# Autodesk Inventor assembly: right_leg
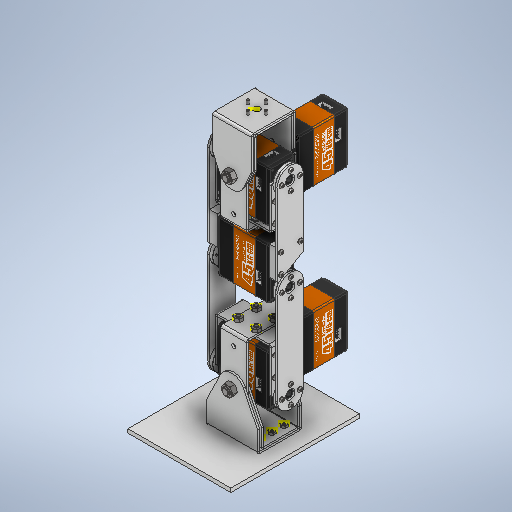
[picture p0: Inventor's stored thumbnail of the model, 512x512]
Saved by Autodesk Inventor 2026.1 (Build 301233000, 233)
## iProperties
Created: 2025-08-03
Part Number: right_leg
Document SubType Name: Assembly
Designer: User
Author: User
## Documents named in this file (29)
- C:\Users\chris\Documents\Inventor\RHp_Humanoid_ver1\Total\right_leg.iam
- C:\Users\chris\Documents\Inventor\RHp_Humanoid_ver1\Part_Body\HTD-45H, Horn (Silver)\HTD-45H\HTD-45H.iam
- C:\Users\chris\Documents\Inventor\RHp_Humanoid_ver1\Part_Leg\Frame\Leg\Left Leg\axis_1_top_frame.ipt
- C:\Users\chris\Documents\Inventor\RHp_Humanoid_ver1\Part_Leg\Frame\Leg\Left Leg\axis_3_bottom_frame.ipt
- C:\Users\chris\Documents\Inventor\RHp_Humanoid_ver1\Part_Leg\Frame\Leg\Left Leg\axis_2_bottom_frame.ipt
- C:\Users\chris\Documents\Inventor\RHp_Humanoid_ver1\Part_Leg\Frame\Leg\Left Leg\axis_1_supplement_frame.ipt
- C:\Users\chris\Documents\Inventor\RHp_Humanoid_ver1\Part_Leg\Frame\Leg\Left Leg\axis_2_4_connector_frame_powered.ipt
- C:\Users\chris\Documents\Inventor\RHp_Humanoid_ver1\Part_Leg\Frame\Leg\Left Leg\axis_2_4_connector_frame_non_powered.ipt
- C:\Users\chris\Documents\Inventor\RHp_Humanoid_ver1\Part_Leg\Frame\Leg\3D_printed_part_powered.ipt
- C:\Users\chris\Documents\Inventor\RHp_Humanoid_ver1\Part_Leg\Frame\Leg\3D_printed_part_non_powered.ipt
- C:\Users\chris\Documents\Inventor\RHp_Humanoid_ver1\Part_Leg\Frame\Leg\Left Leg\axis_4_5_connector_frame_powered.ipt
- C:\Users\chris\Documents\Inventor\RHp_Humanoid_ver1\Part_Leg\Frame\Leg\Left Leg\axis_4_5_connector_frame_non_powered.ipt
- C:\Users\chris\Documents\Inventor\RHp_Humanoid_ver1\Part_Leg\Frame\Leg\Left Leg\axis_5_top_frame.ipt
- C:\Users\chris\Documents\Inventor\RHp_Humanoid_ver1\Part_Leg\Frame\Leg\Left Leg\axis_6_top_frame.ipt
- C:\Users\chris\Documents\Inventor\RHp_Humanoid_ver1\Part_Leg\Frame\Leg\Left Leg\axis_6_bottom_frame(top).ipt
- C:\Users\chris\Documents\Inventor\RHp_Humanoid_ver1\Part_Leg\Frame\Leg\Left Leg\axis_6_bottom_frame(bottom).ipt
- C:\Users\chris\Documents\Inventor\RHp_Humanoid_ver1\Part_Leg\Frame\Leg\Left Leg\axis_6_supplement_frame.ipt
- C:\Users\chris\Documents\Inventor\RHp_Humanoid_ver1\Part_Leg\Bolt, Bearing, Nut, Washer\볼트, 너트\볼트, 너트\M5x10 Bolt.ipt
- C:\Users\chris\Documents\Inventor\RHp_Humanoid_ver1\Part_Leg\Bolt, Bearing, Nut, Washer\볼트, 너트\볼트, 너트\M5 Nylon Nut.ipt
- C:\Users\chris\Documents\Inventor\RHp_Humanoid_ver1\Part_Leg\Bolt, Bearing, Nut, Washer\볼트, 너트\볼트, 너트\M3x6 Bolt.ipt
- C:\Users\chris\Documents\Inventor\RHp_Humanoid_ver1\Part_Leg\Bolt, Bearing, Nut, Washer\볼트, 너트\볼트, 너트\M3 Nut.ipt
- C:\Users\chris\Documents\Inventor\RHp_Humanoid_ver1\Part_Leg\Bolt, Bearing, Nut, Washer\볼트, 너트\볼트, 너트\M2x6 Bolt.ipt
- C:\Users\chris\Documents\Inventor\RHp_Humanoid_ver1\Part_Leg\Bolt, Bearing, Nut, Washer\볼트, 너트\볼트, 너트\M2x4 Bolt.ipt
- C:\Users\chris\Documents\Inventor\RHp_Humanoid_ver1\Part_Leg\Bolt, Bearing, Nut, Washer\볼트, 너트\볼트, 너트\M2x12 Bolt.ipt
- C:\Users\chris\Documents\Inventor\RHp_Humanoid_ver1\Part_Leg\Bolt, Bearing, Nut, Washer\볼트, 너트\볼트, 너트\M2x8접시.ipt
- C:\Users\chris\Documents\Inventor\RHp_Humanoid_ver1\Part_Leg\Bolt, Bearing, Nut, Washer\볼트, 너트\볼트, 너트\M2x45 Bolt.ipt
- C:\Users\chris\Documents\Inventor\RHp_Humanoid_ver1\Part_Leg\HTD-45H, Horn (Silver)\HTD-45H, Horn (Silver)\Horn\Top Horn.ipt
- C:\Users\chris\Documents\Inventor\RHp_Humanoid_ver1\Part_Leg\HTD-45H, Horn (Silver)\HTD-45H, Horn (Silver)\Horn\Bottom Horn.ipt
- C:\Users\chris\Documents\Inventor\RHp_Humanoid_ver1\Part_Leg\Bolt, Bearing, Nut, Washer\M2 Nut.ipt
## Components (132 placed, 28 different names)
1. axis_1_top_frame:1 — Rigid:2, Rigid:7, Rigid:14
2. axis_1_supplement_frame:1 — Rigid:2, Rigid:3, Rigid:4, Rigid:5, Rigid:6, Rigid:8, Rigid:9, Rigid:10, Rigid:11, Rigid:13
3. HTD-45H:3 [sub-assembly] — Rigid:15, Rotational:3
4. Top Horn:2 — Rotational:3, Rigid:17
5. Bottom Horn:2 — Rigid:27
6. axis_2_bottom_frame:1 — Rigid:15, Rigid:16, Rigid:22, Rigid:23, Rigid:24, Rigid:25, Rigid:26, Rigid:28, Rigid:29, Rigid:30, Rigid:31, Rigid:40, Rigid:41, Rigid:42, Rigid:43
7. axis_2_4_connector_frame_powered:1 — Rigid:17, Rigid:18, Rigid:19, Rigid:20, Rigid:21, Rigid:55, Rigid:56, Rigid:57, Rigid:58, Rigid:59, Rigid:60
8. axis_2_4_connector_frame_non_powered:1 — Rigid:27, Rigid:32, Rigid:33, Rigid:50, Rigid:34, Rigid:49, Rigid:51, Rigid:52, Rigid:53
9. HTD-45H:2 [sub-assembly] — Rotational:2, Rigid:12
10. Top Horn:3 — Rotational:2, Rigid:7
11. axis_3_bottom_frame:1 — Rigid:12, Rigid:16, Rigid:35, Rigid:36, Rigid:37, Rigid:38, Rigid:39, Rigid:44, Rigid:45, Rigid:46, Rigid:47
12. HTD-45H:4 [sub-assembly] — Rigid:48, Rigid:54, Rotational:4, Rotational:5
13. Top Horn:4 — Rotational:4, Rigid:61
14. Bottom Horn:4 — Rotational:5, Rigid:66
15. 3D_printed_part_powered:1 — Rigid:54, Rigid:55
16. 3D_printed_part_non_powered:1 — Rigid:48, Rigid:49
17. axis_4_5_connector_frame_powered:1 — Rigid:61, Rigid:62, Rigid:63, Rigid:64, Rigid:65, Rigid:81, Rigid:82, Rigid:83, Rigid:84, Rigid:106
18. axis_4_5_connector_frame_non_powered:1 — Rigid:66, Rigid:67, Rigid:68, Rigid:69, Rigid:70, Rigid:109, Rigid:90, Rigid:91, Rigid:92, Rigid:93
19. HTD-45H:5 [sub-assembly] — Rotational:6, Rotational:7, Rigid:127
20. Top Horn:5 — Rotational:6, Rigid:106
21. Bottom Horn:5 — Rotational:7, Rigid:109
22. axis_5_top_frame:1 — Rigid:72, Rigid:73, Rigid:74, Rigid:75, Rigid:76, Rigid:85, Rigid:86, Rigid:87, Rigid:88, Rigid:89, Rigid:110, Rigid:111, Rigid:112, Rigid:113, Rigid:127
23. HTD-45H:6 [sub-assembly] — Rigid:94, Rotational:8
24. Top Horn:6 — Rotational:8, Rigid:100
25. axis_6_top_frame:1 — Rigid:72, Rigid:77, Rigid:78, Rigid:79, Rigid:80, Rigid:94, Rigid:95, Rigid:96, Rigid:97, Rigid:98, Rigid:99
26. axis_6_supplement_frame:1 — Rigid:101, Rigid:102, Rigid:103, Rigid:104, Rigid:105, Rigid:107, Rigid:121, Rigid:122, Rigid:123, Rigid:124, Rigid:125, Rigid:126
27. axis_6_bottom_frame(top):1 — Rigid:100, Rigid:101, Rigid:108, Rigid:114
28. axis_6_bottom_frame(bottom):1 — Rigid:114, Rigid:115, Rigid:116, Rigid:117, Rigid:118, Rigid:119, Rigid:120
29. M2x4 Bolt:1 — Rigid:81
30. M2x4 Bolt:2 — Rigid:82
31. M2x4 Bolt:3 — Rigid:83
32. M2x4 Bolt:4 — Rigid:84
33. M2x4 Bolt:5 — Rigid:62
34. M2x4 Bolt:6 — Rigid:63
35. M2x4 Bolt:7 — Rigid:64
36. M2x4 Bolt:8 — Rigid:65
37. M2x4 Bolt:9 — Rigid:18
38. M2x4 Bolt:10 — Rigid:19
39. M2x4 Bolt:11 — Rigid:20
40. M2x4 Bolt:12 — Rigid:21
41. M2x4 Bolt:13 — Rigid:90
42. M2x4 Bolt:14 — Rigid:91
43. M2x4 Bolt:15 — Rigid:92
44. M2x4 Bolt:16 — Rigid:93
45. M2x4 Bolt:17 — Rigid:67
46. M2x4 Bolt:18 — Rigid:68
47. M2x4 Bolt:19 — Rigid:69
48. M2x4 Bolt:20 — Rigid:70
49. M2x4 Bolt:21 — Rigid:32
50. M2x4 Bolt:22 — Rigid:33
51. M2x4 Bolt:23 — Rigid:50
52. M2x4 Bolt:24 — Rigid:34
53. M2x6 Bolt:1 — Rigid:85
54. M2x6 Bolt:2 — Rigid:86
55. M2x6 Bolt:3 — Rigid:87
56. M2x6 Bolt:4 — Rigid:88
57. M2x6 Bolt:5 — Rigid:89
58. M2x6 Bolt:6 — Rigid:110
59. M2x6 Bolt:7 — Rigid:111
60. M2x6 Bolt:8 — Rigid:112
61. M2x6 Bolt:9 — Rigid:113
62. M2x6 Bolt:10 — Rigid:95
63. M2x6 Bolt:11 — Rigid:96
64. M2x6 Bolt:12 — Rigid:99
65. M2x6 Bolt:13 — Rigid:97
66. M2x6 Bolt:14 — Rigid:98
67. M2x6 Bolt:15 — Rigid:26
68. M2x6 Bolt:16 — Rigid:25
69. M2x6 Bolt:17 — Rigid:24
70. M2x6 Bolt:18 — Rigid:23
71. M2x6 Bolt:19 — Rigid:22
72. M2x6 Bolt:20 — Rigid:28
73. M2x6 Bolt:21 — Rigid:29
74. M2x6 Bolt:22 — Rigid:30
75. M2x6 Bolt:23 — Rigid:31
76. M2x6 Bolt:24 — Rigid:39
77. M2x6 Bolt:25 — Rigid:38
78. M2x6 Bolt:26 — Rigid:37
79. M2x6 Bolt:27 — Rigid:36
80. M2x6 Bolt:28 — Rigid:35
81. M2x6 Bolt:29 — Rigid:102
82. M2x6 Bolt:30 — Rigid:103
83. M2x6 Bolt:31 — Rigid:104
84. M2x6 Bolt:32 — Rigid:105
85. M2x6 Bolt:33 — Rigid:8
86. M2x6 Bolt:34 — Rigid:9
87. M2x6 Bolt:35 — Rigid:10
88. M2x6 Bolt:36 — Rigid:11
89. M2x6 Bolt:37 — Rigid:4
90. M2x6 Bolt:38 — Rigid:5
91. M2x6 Bolt:39 — Rigid:6
92. M2x6 Bolt:40 — Rigid:3
93. M2x8접시:1 — Rigid:115
94. M2x8접시:2 — Rigid:116
95. M2x8접시:3 — Rigid:117
96. M2x8접시:4 — Rigid:118
97. M2x8접시:5 — Rigid:119
98. M2x8접시:6 — Rigid:120
99. M2x12 Bolt:1 — Rigid:58
100. M2x12 Bolt:2 — Rigid:59
101. M2x12 Bolt:3 — Rigid:60
102. M2x12 Bolt:4 — Rigid:51
103. M2x12 Bolt:5 — Rigid:52
104. M2x12 Bolt:6 — Rigid:53
105. M2x45 Bolt:1 — Rigid:56
106. M2x45 Bolt:2 — Rigid:57
107. M2 Nut:1 — Rigid:121
108. M2 Nut:2 — Rigid:122
109. M2 Nut:3 — Rigid:123
110. M2 Nut:4 — Rigid:124
111. M2 Nut:5 — Rigid:125
112. M2 Nut:6 — Rigid:126
113. M3x6 Bolt:1 — Rigid:40
114. M3x6 Bolt:2 — Rigid:42
115. M3x6 Bolt:3 — Rigid:41
116. M3x6 Bolt:4 — Rigid:43
117. M3x6 Bolt:5 — Rigid:73
118. M3x6 Bolt:6 — Rigid:75
119. M3x6 Bolt:7 — Rigid:74
120. M3x6 Bolt:8 — Rigid:76
121. M3 Nut:1 — Rigid:46
122. M3 Nut:2 — Rigid:44
123. M3 Nut:3 — Rigid:45
124. M3 Nut:4 — Rigid:47
125. M3 Nut:5 — Rigid:77
126. M3 Nut:6 — Rigid:78
127. M3 Nut:7 — Rigid:79
128. M3 Nut:8 — Rigid:80
129. M5x10 Bolt:1 — Rigid:13
130. M5x10 Bolt:4 — Rigid:107
131. M5 Nylon Nut:1 — Rigid:14
132. M5 Nylon Nut:2 — Rigid:108
## Relationships (132: WeldJoint 125, RevoluteJoint 7)
- Rigid:2 [WeldJoint]: axis_1_top_frame:1 ↔ axis_1_supplement_frame:1
- Rigid:3 [WeldJoint]: axis_1_supplement_frame:1 ↔ M2x6 Bolt:40
- Rigid:4 [WeldJoint]: axis_1_supplement_frame:1 ↔ M2x6 Bolt:37
- Rigid:5 [WeldJoint]: axis_1_supplement_frame:1 ↔ M2x6 Bolt:38
- Rigid:6 [WeldJoint]: axis_1_supplement_frame:1 ↔ M2x6 Bolt:39
- Rotational:2 [RevoluteJoint]: HTD-45H:2 ↔ Top Horn:3
- Rigid:7 [WeldJoint]: axis_1_top_frame:1 ↔ Top Horn:3
- Rigid:8 [WeldJoint]: axis_1_supplement_frame:1 ↔ M2x6 Bolt:33
- Rigid:9 [WeldJoint]: axis_1_supplement_frame:1 ↔ M2x6 Bolt:34
- Rigid:10 [WeldJoint]: axis_1_supplement_frame:1 ↔ M2x6 Bolt:35
- Rigid:11 [WeldJoint]: axis_1_supplement_frame:1 ↔ M2x6 Bolt:36
- Rigid:12 [WeldJoint]: HTD-45H:2 ↔ axis_3_bottom_frame:1
- Rigid:13 [WeldJoint]: axis_1_supplement_frame:1 ↔ M5x10 Bolt:1
- Rigid:14 [WeldJoint]: axis_1_top_frame:1 ↔ M5 Nylon Nut:1
- Rigid:15 [WeldJoint]: HTD-45H:3 ↔ axis_2_bottom_frame:1
- Rigid:16 [WeldJoint]: axis_2_bottom_frame:1 ↔ axis_3_bottom_frame:1
- Rotational:3 [RevoluteJoint]: HTD-45H:3 ↔ Top Horn:2
- Rigid:17 [WeldJoint]: Top Horn:2 ↔ axis_2_4_connector_frame_powered:1
- Rigid:18 [WeldJoint]: axis_2_4_connector_frame_powered:1 ↔ M2x4 Bolt:9
- Rigid:19 [WeldJoint]: axis_2_4_connector_frame_powered:1 ↔ M2x4 Bolt:10
- Rigid:20 [WeldJoint]: axis_2_4_connector_frame_powered:1 ↔ M2x4 Bolt:11
- Rigid:21 [WeldJoint]: axis_2_4_connector_frame_powered:1 ↔ M2x4 Bolt:12
- Rigid:22 [WeldJoint]: axis_2_bottom_frame:1 ↔ M2x6 Bolt:19
- Rigid:23 [WeldJoint]: axis_2_bottom_frame:1 ↔ M2x6 Bolt:18
- Rigid:24 [WeldJoint]: axis_2_bottom_frame:1 ↔ M2x6 Bolt:17
- Rigid:25 [WeldJoint]: axis_2_bottom_frame:1 ↔ M2x6 Bolt:16
- Rigid:26 [WeldJoint]: axis_2_bottom_frame:1 ↔ M2x6 Bolt:15
- Rigid:27 [WeldJoint]: Bottom Horn:2 ↔ axis_2_4_connector_frame_non_powered:1
- Rigid:28 [WeldJoint]: axis_2_bottom_frame:1 ↔ M2x6 Bolt:20
- Rigid:29 [WeldJoint]: axis_2_bottom_frame:1 ↔ M2x6 Bolt:21
- Rigid:30 [WeldJoint]: axis_2_bottom_frame:1 ↔ M2x6 Bolt:22
- Rigid:31 [WeldJoint]: axis_2_bottom_frame:1 ↔ M2x6 Bolt:23
- Rigid:32 [WeldJoint]: axis_2_4_connector_frame_non_powered:1 ↔ M2x4 Bolt:21
- Rigid:33 [WeldJoint]: axis_2_4_connector_frame_non_powered:1 ↔ M2x4 Bolt:22
- Rigid:50 [WeldJoint]: axis_2_4_connector_frame_non_powered:1 ↔ M2x4 Bolt:23
- Rigid:34 [WeldJoint]: axis_2_4_connector_frame_non_powered:1 ↔ M2x4 Bolt:24
- Rigid:35 [WeldJoint]: axis_3_bottom_frame:1 ↔ M2x6 Bolt:28
- Rigid:36 [WeldJoint]: axis_3_bottom_frame:1 ↔ M2x6 Bolt:27
- Rigid:37 [WeldJoint]: axis_3_bottom_frame:1 ↔ M2x6 Bolt:26
- Rigid:38 [WeldJoint]: axis_3_bottom_frame:1 ↔ M2x6 Bolt:25
- Rigid:39 [WeldJoint]: axis_3_bottom_frame:1 ↔ M2x6 Bolt:24
- Rigid:40 [WeldJoint]: axis_2_bottom_frame:1 ↔ M3x6 Bolt:1
- Rigid:41 [WeldJoint]: axis_2_bottom_frame:1 ↔ M3x6 Bolt:3
- Rigid:42 [WeldJoint]: axis_2_bottom_frame:1 ↔ M3x6 Bolt:2
- Rigid:43 [WeldJoint]: axis_2_bottom_frame:1 ↔ M3x6 Bolt:4
- Rigid:44 [WeldJoint]: axis_3_bottom_frame:1 ↔ M3 Nut:2
- Rigid:45 [WeldJoint]: axis_3_bottom_frame:1 ↔ M3 Nut:3
- Rigid:46 [WeldJoint]: axis_3_bottom_frame:1 ↔ M3 Nut:1
- Rigid:47 [WeldJoint]: axis_3_bottom_frame:1 ↔ M3 Nut:4
- Rigid:48 [WeldJoint]: HTD-45H:4 ↔ 3D_printed_part_non_powered:1
- Rigid:49 [WeldJoint]: axis_2_4_connector_frame_non_powered:1 ↔ 3D_printed_part_non_powered:1
- Rigid:51 [WeldJoint]: axis_2_4_connector_frame_non_powered:1 ↔ M2x12 Bolt:4
- Rigid:52 [WeldJoint]: axis_2_4_connector_frame_non_powered:1 ↔ M2x12 Bolt:5
- Rigid:53 [WeldJoint]: axis_2_4_connector_frame_non_powered:1 ↔ M2x12 Bolt:6
- Rigid:54 [WeldJoint]: HTD-45H:4 ↔ 3D_printed_part_powered:1
- Rigid:55 [WeldJoint]: axis_2_4_connector_frame_powered:1 ↔ 3D_printed_part_powered:1
- Rigid:56 [WeldJoint]: axis_2_4_connector_frame_powered:1 ↔ M2x45 Bolt:1
- Rigid:57 [WeldJoint]: axis_2_4_connector_frame_powered:1 ↔ M2x45 Bolt:2
- Rigid:58 [WeldJoint]: axis_2_4_connector_frame_powered:1 ↔ M2x12 Bolt:1
- Rigid:59 [WeldJoint]: axis_2_4_connector_frame_powered:1 ↔ M2x12 Bolt:2
- Rigid:60 [WeldJoint]: axis_2_4_connector_frame_powered:1 ↔ M2x12 Bolt:3
- Rotational:4 [RevoluteJoint]: HTD-45H:4 ↔ Top Horn:4
- Rigid:61 [WeldJoint]: Top Horn:4 ↔ axis_4_5_connector_frame_powered:1
- Rigid:62 [WeldJoint]: axis_4_5_connector_frame_powered:1 ↔ M2x4 Bolt:5
- Rigid:63 [WeldJoint]: axis_4_5_connector_frame_powered:1 ↔ M2x4 Bolt:6
- Rigid:64 [WeldJoint]: axis_4_5_connector_frame_powered:1 ↔ M2x4 Bolt:7
- Rigid:65 [WeldJoint]: axis_4_5_connector_frame_powered:1 ↔ M2x4 Bolt:8
- Rotational:5 [RevoluteJoint]: HTD-45H:4 ↔ Bottom Horn:4
- Rigid:66 [WeldJoint]: Bottom Horn:4 ↔ axis_4_5_connector_frame_non_powered:1
- Rigid:67 [WeldJoint]: axis_4_5_connector_frame_non_powered:1 ↔ M2x4 Bolt:17
- Rigid:68 [WeldJoint]: axis_4_5_connector_frame_non_powered:1 ↔ M2x4 Bolt:18
- Rigid:69 [WeldJoint]: axis_4_5_connector_frame_non_powered:1 ↔ M2x4 Bolt:19
- Rigid:70 [WeldJoint]: axis_4_5_connector_frame_non_powered:1 ↔ M2x4 Bolt:20
- Rigid:72 [WeldJoint]: axis_5_top_frame:1 ↔ axis_6_top_frame:1
- Rigid:73 [WeldJoint]: axis_5_top_frame:1 ↔ M3x6 Bolt:5
- Rigid:74 [WeldJoint]: axis_5_top_frame:1 ↔ M3x6 Bolt:7
- Rigid:75 [WeldJoint]: axis_5_top_frame:1 ↔ M3x6 Bolt:6
- Rigid:76 [WeldJoint]: axis_5_top_frame:1 ↔ M3x6 Bolt:8
- Rigid:77 [WeldJoint]: axis_6_top_frame:1 ↔ M3 Nut:5
- Rigid:78 [WeldJoint]: axis_6_top_frame:1 ↔ M3 Nut:6
- Rigid:79 [WeldJoint]: axis_6_top_frame:1 ↔ M3 Nut:7
- Rigid:80 [WeldJoint]: axis_6_top_frame:1 ↔ M3 Nut:8
- Rotational:6 [RevoluteJoint]: HTD-45H:5 ↔ Top Horn:5
- Rigid:81 [WeldJoint]: axis_4_5_connector_frame_powered:1 ↔ M2x4 Bolt:1
- Rigid:82 [WeldJoint]: axis_4_5_connector_frame_powered:1 ↔ M2x4 Bolt:2
- Rigid:83 [WeldJoint]: axis_4_5_connector_frame_powered:1 ↔ M2x4 Bolt:3
- Rigid:84 [WeldJoint]: axis_4_5_connector_frame_powered:1 ↔ M2x4 Bolt:4
- Rigid:85 [WeldJoint]: axis_5_top_frame:1 ↔ M2x6 Bolt:1
- Rigid:86 [WeldJoint]: axis_5_top_frame:1 ↔ M2x6 Bolt:2
- Rigid:87 [WeldJoint]: axis_5_top_frame:1 ↔ M2x6 Bolt:3
- Rigid:88 [WeldJoint]: axis_5_top_frame:1 ↔ M2x6 Bolt:4
- Rigid:89 [WeldJoint]: axis_5_top_frame:1 ↔ M2x6 Bolt:5
- Rigid:90 [WeldJoint]: axis_4_5_connector_frame_non_powered:1 ↔ M2x4 Bolt:13
- Rigid:91 [WeldJoint]: axis_4_5_connector_frame_non_powered:1 ↔ M2x4 Bolt:14
- Rigid:92 [WeldJoint]: axis_4_5_connector_frame_non_powered:1 ↔ M2x4 Bolt:15
- Rigid:93 [WeldJoint]: axis_4_5_connector_frame_non_powered:1 ↔ M2x4 Bolt:16
- Rotational:7 [RevoluteJoint]: HTD-45H:5 ↔ Bottom Horn:5
- Rigid:94 [WeldJoint]: HTD-45H:6 ↔ axis_6_top_frame:1
- Rigid:95 [WeldJoint]: axis_6_top_frame:1 ↔ M2x6 Bolt:10
- Rigid:96 [WeldJoint]: axis_6_top_frame:1 ↔ M2x6 Bolt:11
- Rigid:97 [WeldJoint]: axis_6_top_frame:1 ↔ M2x6 Bolt:13
- Rigid:98 [WeldJoint]: axis_6_top_frame:1 ↔ M2x6 Bolt:14
- Rigid:99 [WeldJoint]: axis_6_top_frame:1 ↔ M2x6 Bolt:12
- Rotational:8 [RevoluteJoint]: HTD-45H:6 ↔ Top Horn:6
- Rigid:100 [WeldJoint]: Top Horn:6 ↔ axis_6_bottom_frame(top):1
- Rigid:101 [WeldJoint]: axis_6_supplement_frame:1 ↔ axis_6_bottom_frame(top):1
- Rigid:102 [WeldJoint]: axis_6_supplement_frame:1 ↔ M2x6 Bolt:29
- Rigid:103 [WeldJoint]: axis_6_supplement_frame:1 ↔ M2x6 Bolt:30
- Rigid:104 [WeldJoint]: axis_6_supplement_frame:1 ↔ M2x6 Bolt:31
- Rigid:105 [WeldJoint]: axis_6_supplement_frame:1 ↔ M2x6 Bolt:32
- Rigid:106 [WeldJoint]: axis_4_5_connector_frame_powered:1 ↔ Top Horn:5
- Rigid:107 [WeldJoint]: axis_6_supplement_frame:1 ↔ M5x10 Bolt:4
- Rigid:108 [WeldJoint]: axis_6_bottom_frame(top):1 ↔ M5 Nylon Nut:2
- Rigid:109 [WeldJoint]: axis_4_5_connector_frame_non_powered:1 ↔ Bottom Horn:5
- Rigid:110 [WeldJoint]: axis_5_top_frame:1 ↔ M2x6 Bolt:6
- Rigid:111 [WeldJoint]: axis_5_top_frame:1 ↔ M2x6 Bolt:7
- Rigid:112 [WeldJoint]: axis_5_top_frame:1 ↔ M2x6 Bolt:8
- Rigid:113 [WeldJoint]: axis_5_top_frame:1 ↔ M2x6 Bolt:9
- Rigid:114 [WeldJoint]: axis_6_bottom_frame(top):1 ↔ axis_6_bottom_frame(bottom):1
- Rigid:115 [WeldJoint]: axis_6_bottom_frame(bottom):1 ↔ M2x8접시:1
- Rigid:116 [WeldJoint]: axis_6_bottom_frame(bottom):1 ↔ M2x8접시:2
- Rigid:117 [WeldJoint]: axis_6_bottom_frame(bottom):1 ↔ M2x8접시:3
- Rigid:118 [WeldJoint]: axis_6_bottom_frame(bottom):1 ↔ M2x8접시:4
- Rigid:119 [WeldJoint]: axis_6_bottom_frame(bottom):1 ↔ M2x8접시:5
- Rigid:120 [WeldJoint]: axis_6_bottom_frame(bottom):1 ↔ M2x8접시:6
- Rigid:121 [WeldJoint]: axis_6_supplement_frame:1 ↔ M2 Nut:1
- Rigid:122 [WeldJoint]: axis_6_supplement_frame:1 ↔ M2 Nut:2
- Rigid:123 [WeldJoint]: axis_6_supplement_frame:1 ↔ M2 Nut:3
- Rigid:124 [WeldJoint]: axis_6_supplement_frame:1 ↔ M2 Nut:4
- Rigid:125 [WeldJoint]: axis_6_supplement_frame:1 ↔ M2 Nut:5
- Rigid:126 [WeldJoint]: axis_6_supplement_frame:1 ↔ M2 Nut:6
- Rigid:127 [WeldJoint]: HTD-45H:5 ↔ axis_5_top_frame:1
